# Autodesk Inventor assembly: Kog test123
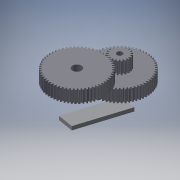
[picture p0: Inventor's stored thumbnail of the model, 180x180]
Saved by Autodesk Inventor 2016 (Build 200138000, 138)
## iProperties
Created: 2018-03-03
Part Number: Kog test123
Document SubType Name: Assembly
Designer: Simon
Author: Simon
## Documents named in this file (4)
- D:\Cad\Gymnasieprojekt\Kog test123.iam
- D:\Cad\Gymnasieprojekt\Spur Gear11.ipt
- D:\Cad\Gymnasieprojekt\Spur Gear21.ipt
- D:\Cad\Gymnasieprojekt\MotorKuggHolder.ipt
## Components (5 placed, 3 different names)
1. Spur Gear1:1 — Insert:2
2. Spur Gear2:1 — Insert:1
3. Spur Gear1:2 — Insert:1
4. Spur Gear2:2 — Insert:2
5. MotorKuggHolder:1
## Relationships (2: Insert 2)
- Insert:1: Spur Gear2:1 ↔ Spur Gear1:2
- Insert:2: Spur Gear1:1 ↔ Spur Gear2:2
